# Autodesk Inventor assembly: Motor Assembly
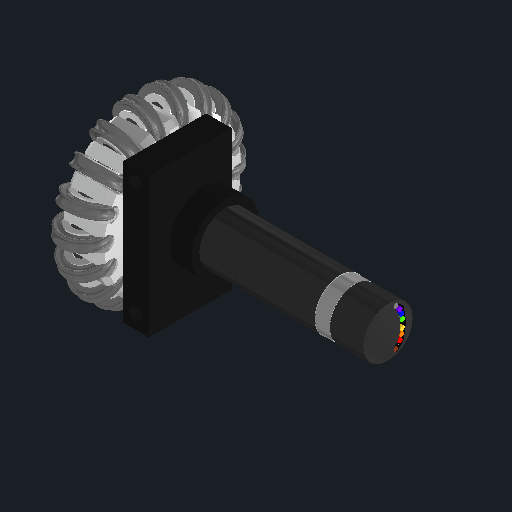
[picture p0: Inventor's stored thumbnail of the model, 512x512]
Saved by Autodesk Inventor 2026.1 (Build 301233020, 233B)
## iProperties
Created: 2025-11-06
Part Number: Motor Assembly
Document SubType Name: Assembly
Designer: Bahaa
Mass: 50.0527 g
Surface Area: 387.288 cm^2
Volume: 40.1669 cm^3
Density: 1.24612 g/cm^3
Author: Bahaa
## Documents named in this file (4)
- C:\Users\Bahaa\Nextcloud2\CAD\25-26\V2\Motor Assembly.iam
- C:\Users\Bahaa\Nextcloud2\CAD\25-26\V2\Motor Bracket.ipt
- C:\Users\Bahaa\Nextcloud2\CAD\25-26\V2\Motoren\Motor.iam
- C:\Users\Bahaa\Nextcloud2\CAD\25-26\V2\RadLWL\RadLWL.iam
## Components (3 placed, 3 different names)
1. Motor Bracket:1 — Mate:1, Mate:6, Mate:7
2. Motor:1 [sub-assembly] — Mate:1, Mate:4, Mate:6, Mate:7
3. RadLWL:1 [sub-assembly] — Mate:4
## Relationships (4: Mate 4)
- Mate:1: Motor Bracket:1 ↔ Motor:1
- Mate:4 (1.5 mm): Motor:1 ↔ RadLWL:1
- Mate:6: Motor Bracket:1 ↔ Motor:1
- Mate:7: Motor Bracket:1 ↔ Motor:1
